# Autodesk Inventor assembly: Assembly
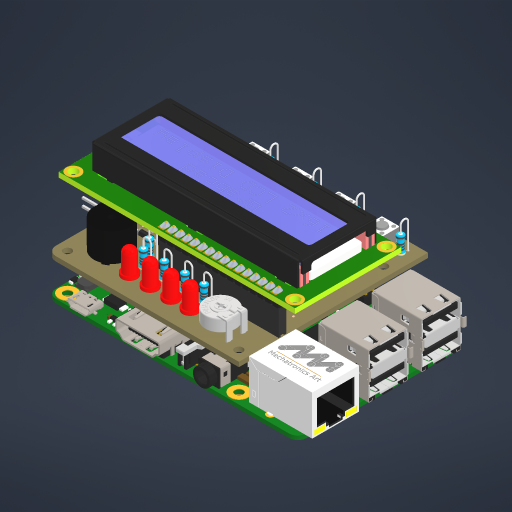
[picture p0: Inventor's stored thumbnail of the model, 512x512]
Saved by Autodesk Inventor 2023 (Build 270158000, 158)
## iProperties
Created: 2022-12-07
Part Number: Assembly
Document SubType Name: Assembly
Designer: Manuel
Author: Manuel
## Documents named in this file (4)
- C:\workspace\Studium\WST\opcua_netzwerk\Entwicklung Knoten\3D Modell\Assembly.iam
- C:\workspace\Studium\WST\opcua_netzwerk\Entwicklung Knoten\3D Modell\ConnectorHead_RPi\ConnectorHead_RPi.iam
- C:\workspace\Studium\WST\opcua_netzwerk\Entwicklung Knoten\3D Modell\Raspberry Pi 3B\Raspberry Pi 3.iam
- C:\workspace\Studium\WST\opcua_netzwerk\Entwicklung Knoten\3D Modell\16x2 LCD Display\LCD.iam
## Components (3 placed, 3 different names)
1. Raspberry Pi 3:1 [sub-assembly] — Fluchtend:1, Fluchtend:2, Passend:1
2. ConnectorHead_RPi:1 [sub-assembly] — Fluchtend:1, Fluchtend:2, Passend:1, Passend:2, Passend:3, Passend:4
3. LCD:1 [sub-assembly] — Passend:2, Passend:3, Passend:4
## Relationships (6: Mate 4, Flush 2)
- Fluchtend:1 [Flush]: Raspberry Pi 3:1 ↔ ConnectorHead_RPi:1
- Fluchtend:2 [Flush]: Raspberry Pi 3:1 ↔ ConnectorHead_RPi:1
- Passend:1 [Mate] (11 mm): Raspberry Pi 3:1 ↔ ConnectorHead_RPi:1
- Passend:2 [Mate]: ConnectorHead_RPi:1 ↔ LCD:1
- Passend:3 [Mate]: ConnectorHead_RPi:1 ↔ LCD:1
- Passend:4 [Mate]: ConnectorHead_RPi:1 ↔ LCD:1
